# Autodesk Inventor assembly: Assembly R2D2
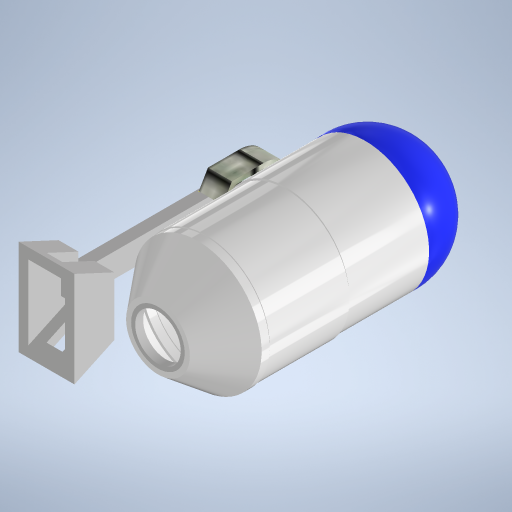
[picture p0: Inventor's stored thumbnail of the model, 512x512]
Saved by Autodesk Inventor 2023 (Build 270158000, 158)
## iProperties
Created: 2022-10-10
Part Number: Assembly R2D2
Document SubType Name: Assembly
Designer: User
Author: User
## Documents named in this file (8)
- C:\Users\User\Videos\R2D2\Partes en 3D\Assembly R2D2.iam
- C:\Users\User\Videos\R2D2\Partes en 3D\Parte media R2D2.ipt
- C:\Users\User\Videos\R2D2\Partes en 3D\Parte baja R2D2.ipt
- C:\Users\User\Videos\R2D2\Partes en 3D\Parte media arriba.ipt
- C:\Users\User\Videos\R2D2\Partes en 3D\Cabeza R2D2.ipt
- C:\Users\User\Videos\R2D2\Partes en 3D\Brazo.ipt
- C:\Users\User\Videos\R2D2\Partes en 3D\Brazo mdf.ipt
- C:\Users\User\Videos\R2D2\Partes en 3D\Pie.ipt
## Components (7 placed, 7 different names)
1. Parte media R2D2:1 — Mate:1, Mate:2
2. Parte baja R2D2:1 — Mate:1
3. Parte media arriba:1 — Mate:2, Mate:3
4. Cabeza R2D2:1 — Mate:3
5. Brazo:1 — Mate:4
6. Brazo mdf:1 — Mate:4
7. Pie:1
## Relationships (4: Mate 4)
- Mate:1: Parte media R2D2:1 ↔ Parte baja R2D2:1
- Mate:2: Parte media R2D2:1 ↔ Parte media arriba:1
- Mate:3: Parte media arriba:1 ↔ Cabeza R2D2:1
- Mate:4: Brazo:1 ↔ Brazo mdf:1
